# Autodesk Inventor assembly: torsion-box-base
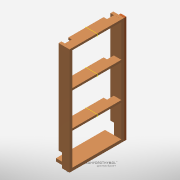
[picture p0: Inventor's stored thumbnail of the model, 180x180]
Saved by Autodesk Inventor 2016 (Build 200138000, 138)
## iProperties
Created: 2015-05-27
Part Number: torsion-box-base
Document SubType Name: Assembly
Designer: as
Mass: 3151.78 g
Surface Area: 7010.96 cm^2
Volume: 5062.26 cm^3
Density: 0.622604 g/cm^3
Author: as
## Documents named in this file (6)
- C:\Users\as\Documents\Inventor\mintplacer-export\torsion-box-base.iam
- C:\Users\as\Documents\Inventor\mintplacer-export\render\MPX-rib.ipt
- C:\Users\as\Documents\Inventor\mintplacer-export\render\MPX-rib2.ipt
- C:\Users\as\Documents\Inventor\mintplacer-export\render\MPX-rib3.ipt
- C:\Users\as\Documents\Inventor\mintplacer-export\MPX-side-spacer.ipt
- C:\Users\as\Documents\Inventor\mintplacer-export\torsion-box-parameters.ipt
## Components (8 placed, 5 different names)
1. MPX-rib3:1 — Mate:2, Flush:3, Flush:4
2. MPX-side-spacer:1 — Mate:3, Flush:5, Flush:6
3. torsion-box-parameters:1
4. MPX-rib2:1 — Flush:1, Flush:2, Mate:1, Mate:2, Flush:3, Flush:4, Mate:3, Flush:5, Flush:6
5. MPX-rib2:2
6. MPX-rib:1 — Flush:1, Flush:2, Mate:1
7. MPX-rib:2
8. MPX-rib:3
## Component patterns: (2 elements, first: MPX-rib2:1), (3 elements, first: MPX-rib:1)
## Relationships (9: Flush 6, Mate 3)
- Flush:1: MPX-rib2:1 ↔ MPX-rib:1
- Flush:2: MPX-rib2:1 ↔ MPX-rib:1
- Mate:1: MPX-rib2:1 ↔ MPX-rib:1
- Mate:2: MPX-rib3:1 ↔ MPX-rib2:1
- Flush:3: MPX-rib3:1 ↔ MPX-rib2:1
- Flush:4: MPX-rib3:1 ↔ MPX-rib2:1
- Mate:3: MPX-side-spacer:1 ↔ MPX-rib2:1
- Flush:5: MPX-side-spacer:1 ↔ MPX-rib2:1
- Flush:6: MPX-side-spacer:1 ↔ MPX-rib2:1
